# Autodesk Inventor assembly: Top-Front-BRace
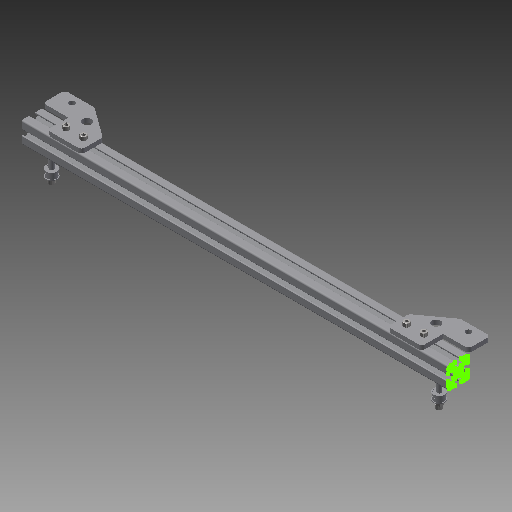
[picture p0: Inventor's stored thumbnail of the model, 512x512]
Saved by Autodesk Inventor 2018 (Build 220112000, 112)
## iProperties
Created: 2016-08-03
Part Number: Top-Front-BRace
Document SubType Name: Assembly
Designer: User
Author: User
## Documents named in this file (6)
- C:\Users\Dan\OneDrive\SL-Inventor\The Beast v1.2 PackandGo\Workspaces\Workspace\Top-Front-BRace.iam
- C:\Users\Dan\OneDrive\SL-Inventor\The Beast v1.2 PackandGo\Workspaces\Workspace\3030 600mm_CPY3.ipt
- C:\Users\Dan\OneDrive\SL-Inventor\The Beast v1.2 PackandGo\Workspaces\Workspace\Y-Idler.iam
- C:\Users\Dan\OneDrive\SL-Inventor\The Beast v1.2 PackandGo\Workspaces\Workspace\Y-Idler2.iam
- C:\Users\Dan\OneDrive\SL-Inventor\The Beast v1.2 PackandGo\Workspaces\Workspace\Front Lead Screw Idler.iam
- C:\Users\Dan\OneDrive\SL-Inventor\The Beast v1.2 PackandGo\Workspaces\Workspace\Front Lead Screw Idler 2.iam
## Components (5 placed, 5 different names)
1. 3030 600mm_CPY3:1 — Mate:3
2. Y-Idler:1 [sub-assembly]
3. Y-Idler2:1 [sub-assembly] — Mate:3
4. Front Lead Screw Idler 2:1 [sub-assembly]
5. Front Lead Screw Idler:1 [sub-assembly]
## Relationships (4: Mate 3, Flush 1)
- [Mate]: 3030 600mm_CPY3:1 ↔ Front Lead Screw Idler 2:1
- [Flush]: 3030 600mm_CPY3:1 ↔ Front Lead Screw Idler:1
- [Mate]: 3030 600mm_CPY3:1 ↔ Front Lead Screw Idler:1
- Mate:3: 3030 600mm_CPY3:1 ↔ Y-Idler2:1
